# Autodesk Inventor assembly: Assembly1
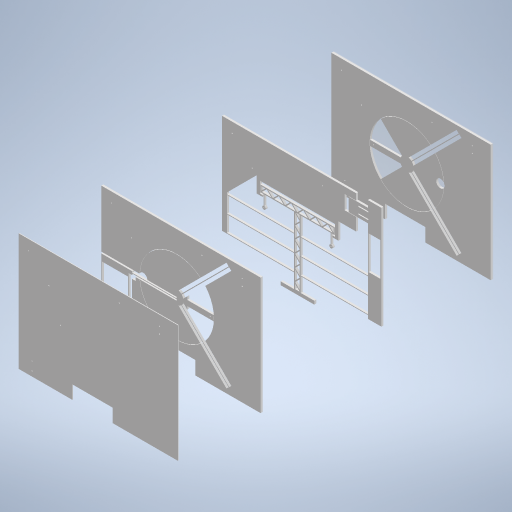
[picture p0: Inventor's stored thumbnail of the model, 512x512]
Saved by Autodesk Inventor 2023 (Build 270158000, 158)
## iProperties
Created: 2023-05-10
Part Number: Assembly1
Document SubType Name: Assembly
Designer: Nathann
Author: Nathann
## Documents named in this file (5)
- C:\Users\Nathann\ClawdDrive\Objet3D\IminaProbe\RoueMDF\Assembly1.iam
- C:\Users\Nathann\ClawdDrive\Objet3D\IminaProbe\RoueMDF\Wheel1.ipt
- C:\Users\Nathann\ClawdDrive\Objet3D\IminaProbe\RoueMDF\Inverter.ipt
- C:\Users\Nathann\ClawdDrive\Objet3D\IminaProbe\RoueMDF\Wheel2.ipt
- C:\Users\Nathann\ClawdDrive\Objet3D\IminaProbe\RoueMDF\Cover.ipt
## Components (5 placed, 4 different names)
1. Wheel1:1 — Flush:1, Flush:2, Flush:3, Flush:4, Flush:5, Flush:6, Mate:1, Mate:2, Flush:8, Flush:9
2. Inverter:1 — Flush:1, Flush:2, Flush:6
3. Wheel2:1 — Flush:3, Flush:4, Flush:5, Flush:7
4. Cover:1 — Flush:7
5. Cover:2 — Flush:8, Flush:9
## Relationships (11: Flush 9, Mate 2)
- Flush:1: Wheel1:1 ↔ Inverter:1
- Flush:2: Wheel1:1 ↔ Inverter:1
- Flush:3: Wheel1:1 ↔ Wheel2:1
- Flush:4: Wheel1:1 ↔ Wheel2:1
- Flush:5: Wheel1:1 ↔ Wheel2:1
- Flush:6: Wheel1:1 ↔ Inverter:1
- Mate:1: Wheel1:1
- Mate:2: Wheel1:1
- Flush:7: Wheel2:1 ↔ Cover:1
- Flush:8: Wheel1:1 ↔ Cover:2
- Flush:9: Wheel1:1 ↔ Cover:2
